# Autodesk Inventor assembly: GE-13032
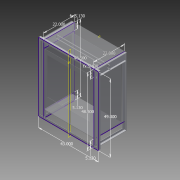
[picture p0: Inventor's stored thumbnail of the model, 180x180]
Saved by Autodesk Inventor 2013 (Build 170138000, 138)
## iProperties
Created: 2013-01-03
Part Number: GE-13032
Document SubType Name: Assembly
Designer: Phillip
Author: Phillip
## Documents named in this file (9)
- C:\Users\Moses\Documents\Inventor\2013 Team 3061 Robot\FIRST Arena 2013\Feeder Goal Station\GE-13032.iam
- C:\Users\Moses\Documents\Inventor\2013 Team 3061 Robot\FIRST Arena 2013\Feeder Goal Station\box_middlegoalLOW.ipt
- C:\Users\Moses\Documents\Inventor\2013 Team 3061 Robot\FIRST Arena 2013\Feeder Goal Station\GE-13053.iam
- C:\Users\Moses\Documents\Inventor\2013 Team 3061 Robot\FIRST Arena 2013\Feeder Goal Station\GE-13054.iam
- C:\Users\Moses\Documents\Inventor\2013 Team 3061 Robot\FIRST Arena 2013\Feeder Goal Station\GE-13056.iam
- C:\Users\Moses\Documents\Inventor\2013 Team 3061 Robot\FIRST Arena 2013\Feeder Goal Station\GE_13030.ipt
- C:\Users\Moses\Documents\Inventor\2013 Team 3061 Robot\FIRST Arena 2013\Feeder Goal Station\GE-13057.ipt
- C:\Users\Moses\Documents\Inventor\2013 Team 3061 Robot\FIRST Arena 2013\Feeder Goal Station\GE-13058.ipt
- C:\Users\Moses\Documents\Inventor\2013 Team 3061 Robot\FIRST Arena 2013\Feeder Goal Station\GE-13059.ipt
## Components (9 placed, 8 different names)
1. box_middlegoalLOW:1 — Mate:4, Mate:8, Mate:9, Flush:1, Mate:11
2. GE-13053:1 [sub-assembly] — Mate:4, Mate:6, Mate:7, Mate:8, Flush:1, Mate:10, Mate:12, Mate:20, Mate:23, Flush:4, Mate:24
3. GE-13054:1 [sub-assembly] — Mate:6, Mate:7, Mate:9, Mate:25, Mate:26
4. GE-13056:1 [sub-assembly] — Mate:10, Mate:11, Mate:12, Mate:13, Mate:14, Angle:1, Tangent:1, Mate:22, Mate:24
5. GE_13030:1 — Mate:13, Mate:14, Mate:17, Mate:20, Flush:2, Flush:3
6. GE_13030:2 — Mate:19, Mate:25, Mate:26
7. GE-13057:1 — Mate:17, Mate:19, Flush:2, Angle:1, Mate:21
8. GE-13058:1 — Flush:3, Mate:21, Tangent:1
9. GE-13059:1 — Mate:22, Mate:23, Flush:4
## Relationships (25: Mate 19, Flush 4, Angle 1, Tangent 1)
- Mate:4: box_middlegoalLOW:1 ↔ GE-13053:1
- Mate:6: GE-13053:1 ↔ GE-13054:1
- Mate:7: GE-13053:1 ↔ GE-13054:1
- Mate:8: box_middlegoalLOW:1 ↔ GE-13053:1
- Mate:9: box_middlegoalLOW:1 ↔ GE-13054:1
- Flush:1 (-133.35 mm): box_middlegoalLOW:1 ↔ GE-13053:1
- Mate:10: GE-13053:1 ↔ GE-13056:1
- Mate:11: box_middlegoalLOW:1 ↔ GE-13056:1
- Mate:12: GE-13053:1 ↔ GE-13056:1
- Mate:13: GE-13056:1 ↔ GE_13030:1
- Mate:14: GE-13056:1 ↔ GE_13030:1
- Mate:17: GE_13030:1 ↔ GE-13057:1
- Mate:19: GE_13030:2 ↔ GE-13057:1
- Mate:20: GE-13053:1 ↔ GE_13030:1
- Flush:2 (36.449 mm): GE_13030:1 ↔ GE-13057:1
- Angle:1 (0 deg): GE-13056:1 ↔ GE-13057:1
- Flush:3 (-36.449 mm): GE_13030:1 ↔ GE-13058:1
- Mate:21: GE-13057:1 ↔ GE-13058:1
- Tangent:1: GE-13056:1 ↔ GE-13058:1
- Mate:22: GE-13056:1 ↔ GE-13059:1
- Mate:23: GE-13053:1 ↔ GE-13059:1
- Flush:4: GE-13053:1 ↔ GE-13059:1
- Mate:24: GE-13053:1 ↔ GE-13056:1
- Mate:25: GE-13054:1 ↔ GE_13030:2
- Mate:26: GE-13054:1 ↔ GE_13030:2
